# Autodesk Inventor assembly: Krabička - dohromady
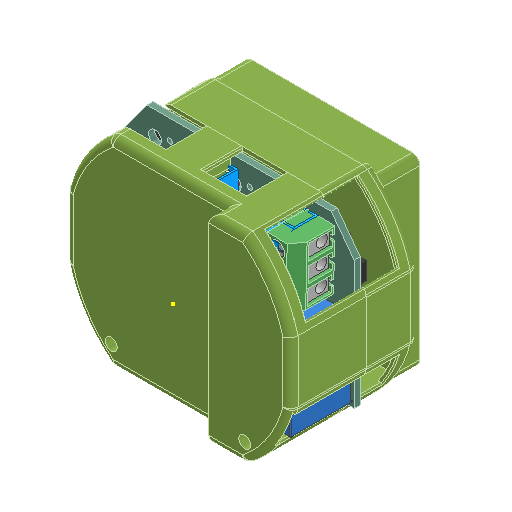
[picture p0: Inventor's stored thumbnail of the model, 512x512]
Saved by Autodesk Inventor 2026.2 (Build 302298010, 298A)
## iProperties
Created: 2026-03-27
Part Number: Krabička - dohromady
Document SubType Name: Weldment
Designer: pokor
Weld Material: Welded Aluminum-6061
Author: pokor
## Documents named in this file (7)
- C:\Users\pokor\Desktop\Inventor 2026\Kryt - soustava.iam
- C:\Users\pokor\Desktop\Krabička - 3D Tisk\Krabička - spodní.ipt
- C:\Users\pokor\Desktop\Krabička - 3D Tisk\Krabička - vrchní.ipt
- C:\Users\pokor\Desktop\DPS - Modul - Úpravy po výrobě\DPS - Modul\DPS - Modul\DPS - Modul.iam
- C:\Users\pokor\Desktop\DPS - Modul - Úpravy po výrobě\Terminal block 5mm\Terminal block 5mm\Terminal block 5mm.ipt
- C:\Program Files\KiCad\9.0\share\kicad\3dmodels\screw-terminal-block-5mm-2.snapshot.17\Screw Terminal Block 5mm 3-way\Screw Terminal Block 5mm 3-way\Screw Terminal Block 5mm 3-way.ipt
- C:\Users\pokor\Downloads\pn532-nfc-rfid-module-v3-kits-1.snapshot.1\PN532_NFC_Assembly\PN532_NFC_Assembly\PN532_NFC_Assembly.ipt
## Components (7 placed, 6 different names)
1. Krabička - vrchní:2 — Mate:15, Mate:16, Mate:17, Mate:18
2. DPS - Modul:2 [sub-assembly]
3. Terminal block 5mm:3
4. Terminal block 5mm:4
5. Screw Terminal Block 5mm 3-way:2
6. Krabička - spodní:3 — Mate:15, Mate:16, Mate:17
7. PN532_NFC_Assembly:1 — Mate:18
## Relationships (12: Mate 10, Tangent 2)
- [Mate]: DPS - Modul:2 ↔ Screw Terminal Block 5mm 3-way:2
- [Tangent]: DPS - Modul:2 ↔ Screw Terminal Block 5mm 3-way:2
- [Tangent]: DPS - Modul:2 ↔ Screw Terminal Block 5mm 3-way:2
- [Mate]: DPS - Modul:2 ↔ Krabička - spodní:3
- [Mate]: DPS - Modul:2 ↔ Krabička - spodní:3
- [Mate]: DPS - Modul:2 ↔ Krabička - spodní:3
- [Mate]: DPS - Modul:2 ↔ Terminal block 5mm:3
- [Mate]: DPS - Modul:2 ↔ Terminal block 5mm:4
- Mate:15: Krabička - vrchní:2 ↔ Krabička - spodní:3
- Mate:16: Krabička - vrchní:2 ↔ Krabička - spodní:3
- Mate:17: Krabička - vrchní:2 ↔ Krabička - spodní:3
- Mate:18: Krabička - vrchní:2 ↔ PN532_NFC_Assembly:1
## Named parameters: d17_d7 = 0 mm, d18_d8 = 0 mm, d19_d12 = 0 mm, d20_d13 = 0 mm, d21_d14 = 0 mm, d22_d15 = 0 mm, d23_d16 = 0 mm, d24_d5 = 0 mm
